# Autodesk Inventor assembly: bottom box with container
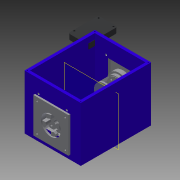
[picture p0: Inventor's stored thumbnail of the model, 180x180]
Saved by Autodesk Inventor 2015 (Build 190159000, 159)
## iProperties
Created: 2014-09-09
Part Number: bottom box with container
Document SubType Name: Assembly
Designer: ericd_000
Author: ericd_000
## Documents named in this file (4)
- C:\Users\ericd_000\Dropbox\GitHub\initial_cad\eric_cad\bottom box with container.iam
- C:\Users\ericd_000\Dropbox\GitHub\initial_cad\eric_cad\bayonet container.ipt
- C:\Users\ericd_000\Dropbox\GitHub\initial_cad\eric_cad\brain box bottom.ipt
- C:\Users\ericd_000\Dropbox\GitHub\initial_cad\eric_cad\bbb brick.ipt
## Components (5 placed, 3 different names)
1. brain box bottom:1 — Rigid:1, Rotational:1, Rotational:2
2. bayonet container:2 — Rigid:1
3. bayonet container:3 — Rotational:1
4. bbb brick:1
5. bayonet container:4 — Rotational:2
## Relationships (3: RevoluteJoint 2, WeldJoint 1)
- Rigid:1 [WeldJoint]: brain box bottom:1 ↔ bayonet container:2
- Rotational:1 [RevoluteJoint]: brain box bottom:1 ↔ bayonet container:3
- Rotational:2 [RevoluteJoint]: brain box bottom:1 ↔ bayonet container:4
